# Autodesk Inventor assembly: Shooter Basic Design
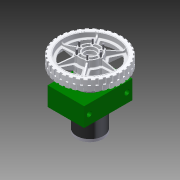
[picture p0: Inventor's stored thumbnail of the model, 180x180]
Saved by Autodesk Inventor 2013 (Build 170138000, 138)
## iProperties
Created: 2013-01-18
Part Number: Shooter Basic Design
Document SubType Name: Assembly
Designer: Naphat
Author: Naphat
## Documents named in this file (6)
- C:\Autodesk\gruntmaster6000-cad\Imported Components\Wheels\Basic Wheel\Shooter Basic Design.iam
- C:\Autodesk\gruntmaster6000-cad\Imported Components\Wheels\6-HiGrip-am-0940\6-HiGrip-am-0940.iam
- C:\Autodesk\gruntmaster6000-cad\Imported Components\Wheels\Basic Wheel\small screw for hub.ipt
- C:\Autodesk\gruntmaster6000-cad\Imported Components\Motors\8mm-key-hub\8mm-key-hub.ipt
- C:\Autodesk\gruntmaster6000-cad\Imported Components\Motors\CIM\CIM Motor.iam
- C:\Autodesk\gruntmaster6000-cad\Imported Components\Motors\CIM Mount\CIM MotorCase.iam
## Components (10 placed, 5 different names)
1. 6-HiGrip-am-0940:1 [sub-assembly] — Mate:40, Mate:57, Mate:58
2. small screw for hub:1 — Mate:42, Mate:43
3. small screw for hub:2 — Mate:48, Mate:49
4. small screw for hub:3 — Mate:52, Mate:53
5. small screw for hub:4 — Mate:46, Mate:47
6. small screw for hub:5 — Mate:50, Mate:51, Mate:57
7. small screw for hub:6 — Mate:44, Mate:45
8. 8mm-key-hub:1 — Mate:40, Mate:42, Mate:43, Mate:44, Mate:45, Mate:46, Mate:47, Mate:48, Mate:49, Mate:50, Mate:51, Mate:52, Mate:53, Mate:55, Mate:56
9. CIM Motor:1 [sub-assembly] — Mate:55, Mate:56, Mate:58, Insert:1
10. CIM MotorCase:1 [sub-assembly] — Insert:1
## Relationships (18: Mate 17, Insert 1)
- Mate:40: 6-HiGrip-am-0940:1 ↔ 8mm-key-hub:1
- Mate:42: small screw for hub:1 ↔ 8mm-key-hub:1
- Mate:43: small screw for hub:1 ↔ 8mm-key-hub:1
- Mate:44: small screw for hub:6 ↔ 8mm-key-hub:1
- Mate:45: small screw for hub:6 ↔ 8mm-key-hub:1
- Mate:46: small screw for hub:4 ↔ 8mm-key-hub:1
- Mate:47: small screw for hub:4 ↔ 8mm-key-hub:1
- Mate:48: small screw for hub:2 ↔ 8mm-key-hub:1
- Mate:49: small screw for hub:2 ↔ 8mm-key-hub:1
- Mate:50: small screw for hub:5 ↔ 8mm-key-hub:1
- Mate:51: small screw for hub:5 ↔ 8mm-key-hub:1
- Mate:52: small screw for hub:3 ↔ 8mm-key-hub:1
- Mate:53: small screw for hub:3 ↔ 8mm-key-hub:1
- Mate:55: 8mm-key-hub:1 ↔ CIM Motor:1
- Mate:56 (12 mm): 8mm-key-hub:1 ↔ CIM Motor:1
- Mate:57: 6-HiGrip-am-0940:1 ↔ small screw for hub:5
- Mate:58: 6-HiGrip-am-0940:1 ↔ CIM Motor:1
- Insert:1: CIM Motor:1 ↔ CIM MotorCase:1
